# Autodesk Inventor assembly: Assembly
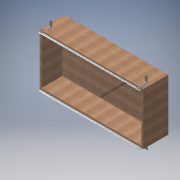
[picture p0: Inventor's stored thumbnail of the model, 180x180]
Saved by Autodesk Inventor 2017 (Build 210142000, 142)
## iProperties
Created: 2016-12-12
Part Number: Assembly
Document SubType Name: Assembly
Designer: umr
Author: umr
## Documents named in this file (18)
- D:\SeniorProject\Models2\BedAssembly\BedAseembly.iam
- D:\SeniorProject\Models2\BedAssembly\Base.ipt
- D:\SeniorProject\Models2\BedAssembly\BedTrack.ipt
- D:\SeniorProject\Models2\BedAssembly\Track Corner Plate.ipt
- D:\SeniorProject\Models2\BedAssembly\Wood Screw 99136A600.ipt
- D:\SeniorProject\Models2\BedAssembly\M5 Screw with Tee Nut.iam
- D:\SeniorProject\Models2\BedAssembly\Track Corner Plate_MIR.ipt
- D:\SeniorProject\Models2\BedAssembly\Wood Screw 99136A600_MIR.ipt
- D:\SeniorProject\Models2\BedAssembly\Wood Screw 99136A600_MIR1.ipt
- D:\SeniorProject\Models2\BedAssembly\Wood Screw 99136A600_MIR_MIR.ipt
- D:\SeniorProject\Models2\BedAssembly\BedTrack_MIR3.ipt
- D:\SeniorProject\Models2\BedAssembly\Track Corner Plate_MIR2.ipt
- D:\SeniorProject\Models2\BedAssembly\Track Corner Plate_MIR_MIR1.ipt
- D:\SeniorProject\Models2\BedAssembly\L_ShapedBracket_100x200x10_ozce.ipt
- D:\SeniorProject\Models2\BedAssembly\L_ShapedBracket_100x200x10_ozce_MIR2.ipt
- D:\SeniorProject\Models2\BedAssembly\L_ShapedBracket_100x200x10_ozce_MIR3.ipt
- D:\SeniorProject\Models2\BedAssembly\L_ShapedBracket_100x200x10_ozce_MIR2_MIR.ipt
- D:\SeniorProject\Models2\BeltMain.ipt
## Components (32 placed, 17 different names)
1. Base:1 — Mate:1, Mate:2, Mate:3, Mate:20, Mate:21, Mate:22, Mate:40, Mate:41, Mate:43, Mate:45, Mate:46, Mate:47, Mate:49, Mate:50, Mate:51, Mate:52, Mate:53
2. BedTrack:1 — Mate:10, Flush:1, Mate:11, Mate:23
3. Track Corner Plate:1 — Mate:1, Mate:2, Mate:3, Cylindrical:1, Cylindrical:2, Mate:4, Mate:5, Mate:6, Mate:7, Mate:8, Mate:9, Flush:1, Mate:11
4. Wood Screw 99136A600:1 — Cylindrical:1
5. Wood Screw 99136A600:2 — Cylindrical:2
6. M5 Screw with Tee Nut:1 [sub-assembly] — Mate:8, Mate:9, Mate:10
7. M5 Screw with Tee Nut:2 [sub-assembly] — Mate:4, Mate:5
8. M5 Screw with Tee Nut:3 [sub-assembly] — Mate:6, Mate:7
9. Track Corner Plate_MIR:1 — Mate:14, Mate:15, Mate:16, Mate:17, Mate:18, Mate:19, Cylindrical:3, Cylindrical:4, Mate:20
10. Wood Screw 99136A600_MIR:1 — Cylindrical:3, Mate:21
11. Wood Screw 99136A600_MIR:2 — Cylindrical:4, Mate:22
12. M5 Screw with Tee Nut:4 [sub-assembly] — Mate:14, Mate:15, Mate:23
13. M5 Screw with Tee Nut:5 [sub-assembly] — Mate:16, Mate:17
14. M5 Screw with Tee Nut:6 [sub-assembly] — Mate:18, Mate:19
15. Wood Screw 99136A600_MIR1:1 — Mate:41
16. Wood Screw 99136A600_MIR1:2 — Mate:40
17. M5 Screw with Tee Nut:7 [sub-assembly]
18. M5 Screw with Tee Nut:8 [sub-assembly]
19. M5 Screw with Tee Nut:9 [sub-assembly]
20. Wood Screw 99136A600_MIR_MIR:1 — Mate:43, Mate:48
21. Wood Screw 99136A600_MIR_MIR:2
22. M5 Screw with Tee Nut:10 [sub-assembly]
23. M5 Screw with Tee Nut:11 [sub-assembly]
24. M5 Screw with Tee Nut:12 [sub-assembly]
25. BedTrack_MIR3:1 — Mate:44, Flush:2, Mate:54, Flush:3
26. Track Corner Plate_MIR2:1 — Mate:44, Flush:2, Mate:45, Mate:46, Mate:47
27. Track Corner Plate_MIR_MIR1:1 — Mate:48, Mate:49, Mate:50
28. L_ShapedBracket_100x200x10_ozce:1 — Mate:51, Mate:52, Mate:53
29. L_ShapedBracket_100x200x10_ozce_MIR2:1
30. L_ShapedBracket_100x200x10_ozce_MIR3:1
31. L_ShapedBracket_100x200x10_ozce_MIR2_MIR:1
32. BeltMain:1 — Mate:54, Flush:3
## Relationships (42: Mate 35, CylindricalJoint 4, Flush 3)
- Mate:1: Base:1 ↔ Track Corner Plate:1
- Mate:2: Base:1 ↔ Track Corner Plate:1
- Mate:3: Base:1 ↔ Track Corner Plate:1
- Cylindrical:1: Track Corner Plate:1 ↔ Wood Screw 99136A600:1
- Cylindrical:2: Track Corner Plate:1 ↔ Wood Screw 99136A600:2
- Mate:4: Track Corner Plate:1 ↔ M5 Screw with Tee Nut:2
- Mate:5: Track Corner Plate:1 ↔ M5 Screw with Tee Nut:2
- Mate:6: Track Corner Plate:1 ↔ M5 Screw with Tee Nut:3
- Mate:7: Track Corner Plate:1 ↔ M5 Screw with Tee Nut:3
- Mate:8: Track Corner Plate:1 ↔ M5 Screw with Tee Nut:1
- Mate:9: Track Corner Plate:1 ↔ M5 Screw with Tee Nut:1
- Mate:10: BedTrack:1 ↔ M5 Screw with Tee Nut:1
- Flush:1 (-8 mm): BedTrack:1 ↔ Track Corner Plate:1
- Mate:11: BedTrack:1 ↔ Track Corner Plate:1
- Mate:14: Track Corner Plate_MIR:1 ↔ M5 Screw with Tee Nut:4
- Mate:15: Track Corner Plate_MIR:1 ↔ M5 Screw with Tee Nut:4
- Mate:16: Track Corner Plate_MIR:1 ↔ M5 Screw with Tee Nut:5
- Mate:17: Track Corner Plate_MIR:1 ↔ M5 Screw with Tee Nut:5
- Mate:18: Track Corner Plate_MIR:1 ↔ M5 Screw with Tee Nut:6
- Mate:19: Track Corner Plate_MIR:1 ↔ M5 Screw with Tee Nut:6
- Cylindrical:3: Track Corner Plate_MIR:1 ↔ Wood Screw 99136A600_MIR:1
- Cylindrical:4: Track Corner Plate_MIR:1 ↔ Wood Screw 99136A600_MIR:2
- Mate:20: Base:1 ↔ Track Corner Plate_MIR:1
- Mate:21: Base:1 ↔ Wood Screw 99136A600_MIR:1
- Mate:22: Base:1 ↔ Wood Screw 99136A600_MIR:2
- Mate:23: BedTrack:1 ↔ M5 Screw with Tee Nut:4
- Mate:40: Base:1 ↔ Wood Screw 99136A600_MIR1:2
- Mate:41: Base:1 ↔ Wood Screw 99136A600_MIR1:1
- Mate:43: Base:1 ↔ Wood Screw 99136A600_MIR_MIR:1
- Mate:44: BedTrack_MIR3:1 ↔ Track Corner Plate_MIR2:1
- Flush:2 (-8 mm): BedTrack_MIR3:1 ↔ Track Corner Plate_MIR2:1
- Mate:45: Base:1 ↔ Track Corner Plate_MIR2:1
- Mate:46: Base:1 ↔ Track Corner Plate_MIR2:1
- Mate:47: Base:1 ↔ Track Corner Plate_MIR2:1
- Mate:48: Wood Screw 99136A600_MIR_MIR:1 ↔ Track Corner Plate_MIR_MIR1:1
- Mate:49: Base:1 ↔ Track Corner Plate_MIR_MIR1:1
- Mate:50: Base:1 ↔ Track Corner Plate_MIR_MIR1:1
- Mate:51: Base:1 ↔ L_ShapedBracket_100x200x10_ozce:1
- Mate:52: Base:1 ↔ L_ShapedBracket_100x200x10_ozce:1
- Mate:53: Base:1 ↔ L_ShapedBracket_100x200x10_ozce:1
- Mate:54: BedTrack_MIR3:1 ↔ BeltMain:1
- Flush:3: BedTrack_MIR3:1 ↔ BeltMain:1
